# Autodesk Inventor assembly: Ajedrez2
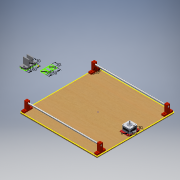
[picture p0: Inventor's stored thumbnail of the model, 180x180]
Saved by Autodesk Inventor 2019 (Build 230136000, 136)
## iProperties
Created: 2019-08-18
Part Number: Ajedrez2
Document SubType Name: Assembly
Designer: Bruno
Author: Bruno
## Documents named in this file (6)
- C:\Users\Bruno\Stuff\Ajedrez2\Ajedrez2.iam
- C:\Users\Bruno\Stuff\Ajedrez2\Floor.ipt
- C:\Users\Bruno\Stuff\Ajedrez2\XRodClamp.ipt
- C:\Users\Bruno\Stuff\Ajedrez2\XRod.ipt
- C:\Users\Bruno\Stuff\Ajedrez2\XMotor.iam
- C:\Users\Bruno\Stuff\Ajedrez2\XPulley.iam
## Components (9 placed, 5 different names)
1. Floor:1 — Rigid:1, Rigid:2, Rigid:3, Rigid:4, Rigid:7
2. XRodClamp:1 — Rigid:1, Rigid:5
3. XRodClamp:2 — Rigid:2
4. XRodClamp:3 — Rigid:3, Rigid:6
5. XRodClamp:4 — Rigid:4
6. XRod:1 — Rigid:5
7. XRod:2 — Rigid:6
8. XMotor:1 [sub-assembly] — Rigid:7
9. XPulley:1 [sub-assembly]
## Relationships (7: WeldJoint 7)
- Rigid:1 [WeldJoint]: Floor:1 ↔ XRodClamp:1
- Rigid:2 [WeldJoint]: Floor:1 ↔ XRodClamp:2
- Rigid:3 [WeldJoint]: Floor:1 ↔ XRodClamp:3
- Rigid:4 [WeldJoint]: Floor:1 ↔ XRodClamp:4
- Rigid:5 [WeldJoint]: XRodClamp:1 ↔ XRod:1
- Rigid:6 [WeldJoint]: XRodClamp:3 ↔ XRod:2
- Rigid:7 [WeldJoint]: Floor:1 ↔ XMotor:1
